# Autodesk Inventor assembly: Omni Wheel
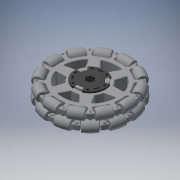
[picture p0: Inventor's stored thumbnail of the model, 180x180]
Saved by Autodesk Inventor 2018 (Build 220112000, 112)
## iProperties
Created: 2018-01-27
Part Number: Omni Wheel
Document SubType Name: Assembly
Designer: S-2512711
Author: S-2512711
## Documents named in this file (4)
- C:\Users\S-2512711\Desktop\Drivebase 2018 Files Final Kinda\Drivebase 2018 Files Final Kinda\Drivebase 2018 Files 2\Drivebase 2018 Files 2\Omni Wheel.iam
- C:\Users\S-2512711\Desktop\Drivebase 2018 Files Final Kinda\Drivebase 2018 Files Final Kinda\Drivebase 2018 Files 2\Drivebase 2018 Files 2\6_Omni-Directional_Wheel_217-2585.ipt
- C:\Users\S-2512711\Desktop\Drivebase 2018 Files Final Kinda\Drivebase 2018 Files Final Kinda\Drivebase 2018 Files 2\Drivebase 2018 Files 2\1_2_Hex_Bore_Aluminum_VersaHub_217-2592.ipt
- C:\Users\S-2512711\Desktop\Drivebase 2018 Files Final Kinda\Drivebase 2018 Files Final Kinda\Drivebase 2018 Files 2\Drivebase 2018 Files 2\1_2_Hex_Bore_Plastic_VersaHub_217-4009.ipt
## Components (3 placed, 3 different names)
1. 6_Omni-Directional_Wheel_217-2585:1 — Mate:1, Mate:2, Rotation:1, Mate:6, Mate:7, Mate:8, Mate:9
2. 1_2_Hex_Bore_Aluminum_VersaHub_217-2592:1 — Mate:7, Mate:8, Mate:9
3. 1_2_Hex_Bore_Plastic_VersaHub_217-4009:1 — Mate:1, Mate:2, Rotation:1, Mate:6
## Relationships (7: Mate 6, RelateRotation 1)
- Mate:1: 6_Omni-Directional_Wheel_217-2585:1 ↔ 1_2_Hex_Bore_Plastic_VersaHub_217-4009:1
- Mate:2: 6_Omni-Directional_Wheel_217-2585:1 ↔ 1_2_Hex_Bore_Plastic_VersaHub_217-4009:1
- Rotation:1 [RelateRotation] (1 ul): 6_Omni-Directional_Wheel_217-2585:1 ↔ 1_2_Hex_Bore_Plastic_VersaHub_217-4009:1
- Mate:6: 6_Omni-Directional_Wheel_217-2585:1 ↔ 1_2_Hex_Bore_Plastic_VersaHub_217-4009:1
- Mate:7: 6_Omni-Directional_Wheel_217-2585:1 ↔ 1_2_Hex_Bore_Aluminum_VersaHub_217-2592:1
- Mate:8: 6_Omni-Directional_Wheel_217-2585:1 ↔ 1_2_Hex_Bore_Aluminum_VersaHub_217-2592:1
- Mate:9: 6_Omni-Directional_Wheel_217-2585:1 ↔ 1_2_Hex_Bore_Aluminum_VersaHub_217-2592:1
